# Autodesk Inventor assembly: demo_1
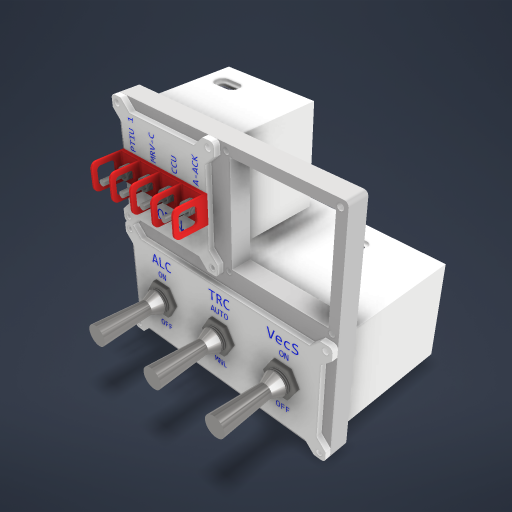
[picture p0: Inventor's stored thumbnail of the model, 512x512]
Saved by Autodesk Inventor 2024 (Build 280153000, 153)
## iProperties
Created: 2026-05-08
Part Number: demo_1
Document SubType Name: Assembly
Designer: schar
Author: schar
## Documents named in this file (4)
- C:\Users\schar\Desktop\MHIPS\models\racks\assembled\demo_1.iam
- C:\Users\schar\Desktop\MHIPS\models\tiles\2x1\lvl202x01_t\lvl202x01.iam
- C:\Users\schar\Desktop\MHIPS\models\tiles\1x1\lvl301x01_4t\1x1_asm_main.iam
- C:\Users\schar\Desktop\MHIPS\models\racks\frames\frame_demo_2x2_xyxx.ipt
## Components (3 placed, 3 different names)
1. lvl202x01:1 [sub-assembly] — Mate:1, Flush:1, Flush:2
2. 1x1_asm_main:1 [sub-assembly] — Mate:1, Flush:1, Flush:2, Flush:3
3. frame_demo_2x2_xyxx:1 — Flush:3
## Relationships (4: Flush 3, Mate 1)
- Mate:1: lvl202x01:1 ↔ 1x1_asm_main:1
- Flush:1: lvl202x01:1 ↔ 1x1_asm_main:1
- Flush:2: lvl202x01:1 ↔ 1x1_asm_main:1
- Flush:3: 1x1_asm_main:1 ↔ frame_demo_2x2_xyxx:1
